# Autodesk Inventor assembly: Chassis
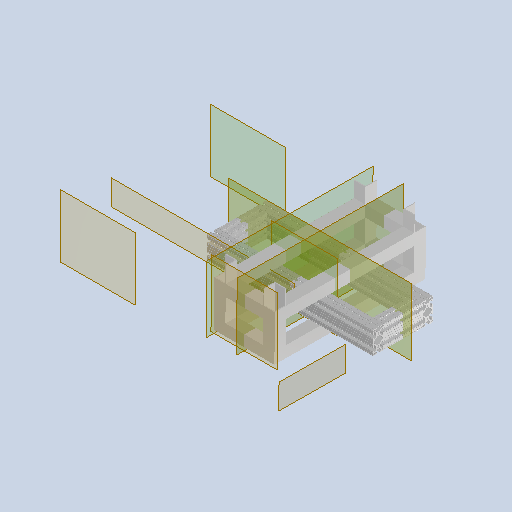
[picture p0: Inventor's stored thumbnail of the model, 512x512]
Saved by Autodesk Inventor 2023 (Build 270158000, 158)
## iProperties
Created: 2022-04-29
Part Number: Chassis
Document SubType Name: Assembly
Designer: Nebil Oumer
Mass: 8270.51 g
Surface Area: 16474 cm^2
Volume: 3063.15 cm^3
Density: 2.7 g/cm^3
Author: Nebil Oumer
## Documents named in this file (4)
- C:\Users\seene\Desktop\Stony Brook\SBRT\RoboRescue\Chassis\Frame\Chassis.iam
- C:\Users\seene\Desktop\Stony Brook\SBRT\RoboRescue\Chassis\Frame\testRoboRescue_Chassis_Frame.iam
- RoboRescue_Chassis_Frame.iam
- C:\Users\seene\Desktop\Stony Brook\SBRT\RoboRescue\Chassis\Frame\DTConnetor-8020.iam
## Components (2 placed, 2 different names)
1. RoboRescue_Chassis_Frame:1 [sub-assembly] — Mate:1, Flush:3, Flush:4, Symmetry:3, Symmetry:4
2. DTConnetor-8020:1 [sub-assembly] — Mate:1, Flush:1, Symmetry:1, Flush:2, Symmetry:2
## Relationships (11: Flush 4, Symmetry 4, Mate 3)
- Mate:1: RoboRescue_Chassis_Frame:1 ↔ DTConnetor-8020:1
- Flush:1: DTConnetor-8020:1
- Symmetry:1: DTConnetor-8020:1
- Flush:2: DTConnetor-8020:1
- Symmetry:2: DTConnetor-8020:1
- Flush:3: RoboRescue_Chassis_Frame:1
- Flush:4: RoboRescue_Chassis_Frame:1
- Symmetry:3: RoboRescue_Chassis_Frame:1
- Symmetry:4: RoboRescue_Chassis_Frame:1
- Mate:2
- Mate:3
